# Autodesk Inventor assembly: Worm
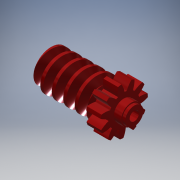
[picture p0: Inventor's stored thumbnail of the model, 180x180]
Saved by Autodesk Inventor 2019.1 (Build 231200000, 200)
## iProperties
Created: 2018-11-21
Part Number: Worm
Material: Generisch
Document SubType Name: Assembly
Designer: JochenAlt
Author: JochenAlt
## Documents named in this file (4)
- D:\Projects\Ondine\CAD\Leg\Worm.iam
- D:\Projects\Ondine\CAD\Leg\Schnecke\Schnecke1.ipt
- D:\Projects\Ondine\CAD\Leg\WormAxis.ipt
- D:\Projects\Ondine\CAD\Leg\Barrel\Stirnzahnrad11.ipt
## Components (3 placed, 3 different names)
1. Schnecke:1 — Drehung:1, Passend:14, Passend:15, Passend:16, Passend:17
2. Stirnzahnrad1:1 — Drehung:1, Passend:14, Passend:15
3. WormAxis:1 — Passend:16, Passend:17
## Relationships (5: Mate 4, RelateRotation 1)
- Drehung:1 [RelateRotation] (1 ul): Schnecke:1 ↔ Stirnzahnrad1:1
- Passend:14 [Mate]: Schnecke:1 ↔ Stirnzahnrad1:1
- Passend:15 [Mate]: Schnecke:1 ↔ Stirnzahnrad1:1
- Passend:16 [Mate]: Schnecke:1 ↔ WormAxis:1
- Passend:17 [Mate] (3 mm): Schnecke:1 ↔ WormAxis:1
